# Autodesk Inventor assembly: Fixture Assembly
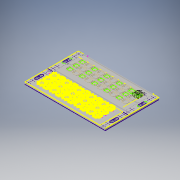
[picture p0: Inventor's stored thumbnail of the model, 180x180]
Saved by Autodesk Inventor 2016 (Build 200138000, 138)
## iProperties
Created: 2016-04-08
Part Number: Fixture Assembly
Document SubType Name: Assembly
Designer: Sam Clay
Author: Sam Clay
## Documents named in this file (6)
- Z:\enclosure\inventor\Fixture Assembly.iam
- Z:\enclosure\inventor\Fixture Base.ipt
- Z:\enclosure\inventor\Case Top.ipt
- Z:\enclosure\inventor\Case Bottom.ipt
- Z:\enclosure\inventor\Case Top Fixture.ipt
- Z:\enclosure\inventor\Case Bottom Fixture.ipt
## Components (61 placed, 5 different names)
1. Fixture Base:1 — Planar:6, Mate:4, Mate:5, Bottom contour planar, Angle:1
2. Case Bottom:1 — Planar:6, Mate top pocket shell, Mate side pocket shell
3. Case Bottom:2
4. Case Bottom:3
5. Case Bottom:4
6. Case Bottom:5
7. Case Bottom:6
8. Case Bottom:7
9. Case Bottom:8
10. Case Bottom:9
11. Case Bottom:10
12. Case Bottom:11
13. Case Bottom:12
14. Case Bottom:13
15. Case Bottom:14
16. Case Bottom:15
17. Case Top:2 — Mate:4, Mate:5, Mate side pocket shell, Mate top pocket shell
18. Case Top:3
19. Case Top:4
20. Case Top:5
21. Case Top:6
22. Case Top:7
23. Case Top:8
24. Case Top:9
25. Case Top:10
26. Case Top:11
27. Case Top:12
28. Case Top:13
29. Case Top:14
30. Case Top:15
31. Case Top:16
32. Case Top Fixture:1 — Mate:8
33. Case Top Fixture:2
34. Case Top Fixture:3
35. Case Top Fixture:4
36. Case Top Fixture:5
37. Case Top Fixture:6
38. Case Top Fixture:7
39. Case Top Fixture:8
40. Case Top Fixture:9
41. Case Top Fixture:10
42. Case Top Fixture:11
43. Case Top Fixture:12
44. Case Top Fixture:13
45. Case Top Fixture:14
46. Case Top Fixture:15
47. Case Bottom Fixture:1 — Bottom contour planar, Angle:1, Mate:8
48. Case Bottom Fixture:2
49. Case Bottom Fixture:3
50. Case Bottom Fixture:4
51. Case Bottom Fixture:5
52. Case Bottom Fixture:6
53. Case Bottom Fixture:7
54. Case Bottom Fixture:8
55. Case Bottom Fixture:9
56. Case Bottom Fixture:10
57. Case Bottom Fixture:11
58. Case Bottom Fixture:12
59. Case Bottom Fixture:13
60. Case Bottom Fixture:14
61. Case Bottom Fixture:15
## Component patterns: (15 elements, first: Case Bottom:1), (15 elements, first: Case Top:2), (15 elements, first: Case Top Fixture:1), (15 elements, first: Case Bottom Fixture:1)
## Relationships (8: Mate 5, PlanarJoint 2, Angle 1)
- Planar:6: Fixture Base:1 ↔ Case Bottom:1
- Mate:4 (1.27 mm): Fixture Base:1 ↔ Case Top:2
- Mate:5 (6.604 mm): Fixture Base:1 ↔ Case Top:2
- Mate top pocket shell: Case Bottom:1 ↔ Case Top:2
- Mate side pocket shell (6.604 mm): Case Bottom:1 ↔ Case Top:2
- Bottom contour planar [PlanarJoint] (16.51 mm): Fixture Base:1 ↔ Case Bottom Fixture:1
- Angle:1 (0 deg): Fixture Base:1 ↔ Case Bottom Fixture:1
- Mate:8 (6.604 mm): Case Top Fixture:1 ↔ Case Bottom Fixture:1
